# Autodesk Inventor assembly: DriveTrain Wheel - one side
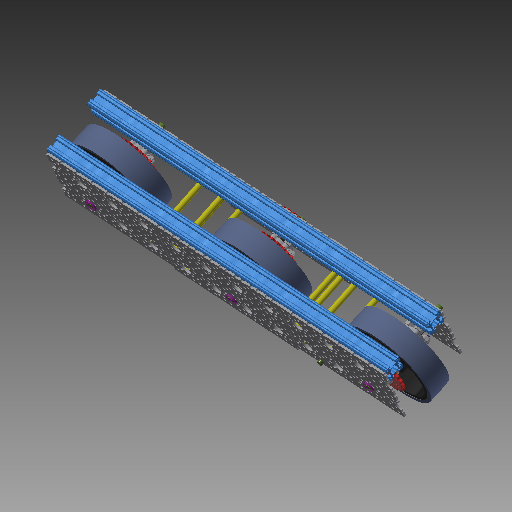
[picture p0: Inventor's stored thumbnail of the model, 512x512]
Saved by Autodesk Inventor 2018 (Build 220112000, 112)
## iProperties
Created: 2017-11-05
Part Number: DriveTrain Wheel - one side
Document SubType Name: Assembly
Designer: ball
Author: ball
## Documents named in this file (11)
- C:\FTC\2017Robot\DriveTrain Wheel - one side.iam
- C:\FTC\2017Robot\DriveTrainSide.iam
- C:\FTC\2017Robot\wheel 2 sprocket.iam
- C:\FTC\2017Robot\wheel 1 sprocket inner.iam
- C:\FTC\2017Robot\wheel 1 sprocket outer.iam
- C:\FTC\Actobotics\633 parts\633150.ipt
- C:\FTC\Actobotics\634 parts\634080.ipt
- C:\FTC\Actobotics\633 parts\633104.ipt
- C:\FTC\Actobotics\545 parts\545619 assembly.ipt
- C:\FTC\Actobotics\615 parts\615106.ipt
- C:\FTC\Actobotics\632 parts\632108.ipt
## Components (20 placed, 10 different names)
1. DriveTrainSide:2 [sub-assembly] — Flush:1, Flush:2, Mate:1, Mate:6, Mate:27, Flush:5, Mate:36, Mate:37
2. DriveTrainSide:3 [sub-assembly] — Flush:1, Flush:2, Mate:1, Mate:2, Mate:3, Mate:4, Mate:5, Mate:7, Mate:8, Mate:9, Mate:10, Mate:11, Mate:12, Mate:13, Mate:14, Mate:15, Mate:16, Mate:17, Mate:18, Mate:20, Mate:21, Mate:22, Mate:23, Mate:24, Mate:28, Mate:29, Mate:30
3. wheel 1 sprocket inner:1 [sub-assembly] — Mate:2, Mate:3
4. wheel 2 sprocket:2 [sub-assembly] — Mate:4, Mate:5
5. wheel 1 sprocket outer:1 [sub-assembly] — Mate:6, Mate:24
6. 633150:1 — Mate:11, Mate:12
7. 633150:2 — Mate:13, Mate:14
8. 633150:3 — Mate:9, Mate:10
9. 633150:4 — Mate:7, Mate:8
10. 633150:5 — Mate:15, Mate:16
11. 633150:6 — Mate:20, Mate:23
12. 633150:7 — Mate:17, Mate:18
13. 633150:8 — Mate:21, Mate:22
14. 634080:3
15. 634080:2
16. 634080:1 — Mate:27, Flush:5
17. 633104:1 — Mate:28, Mate:29, Mate:31
18. 545619 assembly:1 — Mate:30, Mate:31, Mate:32, Mate:33, Mate:34, Mate:35
19. 615106:1 — Mate:32, Mate:33, Mate:34, Mate:35
20. 632108:1 — Mate:36, Mate:37
## Relationships (41: Mate 36, Flush 5)
- Flush:1: DriveTrainSide:2 ↔ DriveTrainSide:3
- Flush:2: DriveTrainSide:2 ↔ DriveTrainSide:3
- Mate:1 (76.2 mm): DriveTrainSide:2 ↔ DriveTrainSide:3
- Mate:2: DriveTrainSide:3 ↔ wheel 1 sprocket inner:1
- Mate:3: DriveTrainSide:3 ↔ wheel 1 sprocket inner:1
- Mate:4: DriveTrainSide:3 ↔ wheel 2 sprocket:2
- Mate:5: DriveTrainSide:3 ↔ wheel 2 sprocket:2
- Mate:6: DriveTrainSide:2 ↔ wheel 1 sprocket outer:1
- Mate:7: DriveTrainSide:3 ↔ 633150:4
- Mate:8: DriveTrainSide:3 ↔ 633150:4
- Mate:9: DriveTrainSide:3 ↔ 633150:3
- Mate:10: DriveTrainSide:3 ↔ 633150:3
- Mate:11: DriveTrainSide:3 ↔ 633150:1
- Mate:12: DriveTrainSide:3 ↔ 633150:1
- Mate:13: DriveTrainSide:3 ↔ 633150:2
- Mate:14: DriveTrainSide:3 ↔ 633150:2
- Mate:15: DriveTrainSide:3 ↔ 633150:5
- Mate:16: DriveTrainSide:3 ↔ 633150:5
- Mate:17: DriveTrainSide:3 ↔ 633150:7
- Mate:18: DriveTrainSide:3 ↔ 633150:7
- Mate:20: DriveTrainSide:3 ↔ 633150:6
- Mate:21: DriveTrainSide:3 ↔ 633150:8
- Mate:22: DriveTrainSide:3 ↔ 633150:8
- Mate:23: DriveTrainSide:3 ↔ 633150:6
- Mate:24: DriveTrainSide:3 ↔ wheel 1 sprocket outer:1
- [Mate]: DriveTrainSide:2 ↔ 634080:3
- [Flush]: DriveTrainSide:2 ↔ 634080:3
- [Mate]: DriveTrainSide:2 ↔ 634080:2
- [Flush]: DriveTrainSide:2 ↔ 634080:2
- Mate:27: DriveTrainSide:2 ↔ 634080:1
- Flush:5: DriveTrainSide:2 ↔ 634080:1
- Mate:28: DriveTrainSide:3 ↔ 633104:1
- Mate:29: DriveTrainSide:3 ↔ 633104:1
- Mate:30: DriveTrainSide:3 ↔ 545619 assembly:1
- Mate:31: 633104:1 ↔ 545619 assembly:1
- Mate:32: 545619 assembly:1 ↔ 615106:1
- Mate:33: 545619 assembly:1 ↔ 615106:1
- Mate:34: 545619 assembly:1 ↔ 615106:1
- Mate:35: 545619 assembly:1 ↔ 615106:1
- Mate:36: DriveTrainSide:2 ↔ 632108:1
- Mate:37: DriveTrainSide:2 ↔ 632108:1
